# Autodesk Inventor assembly: 8 inch mecanum with toughbox (Bottom left)
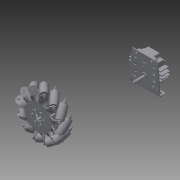
[picture p0: Inventor's stored thumbnail of the model, 180x180]
Saved by Autodesk Inventor 2014 (Build 180170000, 170)
## iProperties
Created: 2015-01-10
Part Number: 8 inch mecanum with toughbox (Bottom left)
Document SubType Name: Assembly
Designer: student
Author: student
## Documents named in this file (4)
- C:\Users\student\Documents\Inventor\2015 Recycle Rush\8 inch mecanum with toughbox (Bottom left).iam
- C:\Users\student\Documents\Inventor\Dillon And Justin\Derived Right Mecanum.ipt
- C:\Users\student\Documents\Inventor\2015 Recycle Rush\am-0077a-500 Key Hub r2.ipt
- C:\Users\student\Documents\Inventor\2015 Recycle Rush\Derived Toughbox mini.ipt
## Components (3 placed, 3 different names)
1. Derived Right Mecanum:1 — Mate:1, Mate:2, Mate:3
2. am-0077a-500 Key Hub r2:2 — Mate:1, Mate:2, Mate:3
3. Derived Toughbox mini:1
## Relationships (3: Mate 3)
- Mate:1: Derived Right Mecanum:1 ↔ am-0077a-500 Key Hub r2:2
- Mate:2: Derived Right Mecanum:1 ↔ am-0077a-500 Key Hub r2:2
- Mate:3: Derived Right Mecanum:1 ↔ am-0077a-500 Key Hub r2:2
